# Autodesk Inventor assembly: inner
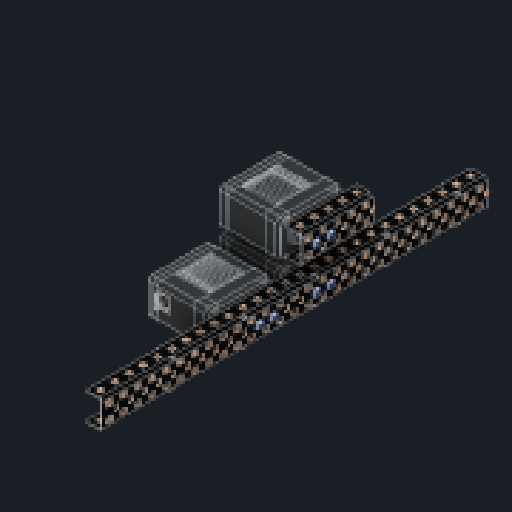
[picture p0: Inventor's stored thumbnail of the model, 512x512]
Saved by Autodesk Inventor 2024 (Build 280153000, 153)
## iProperties
Created: 2024-03-11
Part Number: inner
Document SubType Name: Assembly
Designer: Averey Ku
Author: Averey Ku
## Documents named in this file (17)
- D:\vex_robotics\hardware\cad\eca\chassis\drivebay\inner.iam
- D:\vex_robotics\hardware\cad\VEX-CAD-Inventor-1.41\Structure\C Channel\Aluminum 1x2x1\Alu C 1x2x1x27.ipt
- D:\vex_robotics\hardware\cad\VEX-CAD-Inventor-1.41\Structure\C Channel\Aluminum 1x2x1\Alu C 1x2x1x5.ipt
- D:\vex_robotics\hardware\cad\VEX-CAD-Inventor-1.41\Electronics\Motors with Screws\SteelM-StarS.iam
- D:\vex_robotics\hardware\cad\VEX-CAD-Inventor-1.41\Electronics\Motors with Screws.iam
- D:\vex_robotics\hardware\cad\VEX-CAD-Inventor-1.41\Structure\Hardware\Nut Thin Nylock.ipt
- D:\vex_robotics\hardware\cad\VEX-CAD-Inventor-1.41\Structure\Hardware\Screw Steel - Star\SScrew Star Smooth 1.500.ipt
- D:\vex_robotics\hardware\cad\VEX-CAD-Inventor-1.41\Structure\Hardware\Screw Steel - Star.ipt
- D:\vex_robotics\hardware\cad\VEX-CAD-Inventor-1.41\Structure\Standoff\Standoff .50.ipt
- D:\vex_robotics\hardware\cad\VEX-CAD-Inventor-1.41\Structure\Standoff.ipt
- D:\vex_robotics\hardware\cad\VEX-CAD-Inventor-1.41\Structure\Hardware\Screw Steel - Star\SScrew Star Smooth 1.250.ipt
- D:\vex_robotics\hardware\cad\VEX-CAD-Inventor-1.41\Motion\Spacers\Spacer Nylon .500 OD\NSpacer Black .500 OD x .500.ipt
- D:\vex_robotics\hardware\cad\VEX-CAD-Inventor-1.41\Motion\Spacers\Spacer Nylon .500 OD.ipt
- D:\vex_robotics\hardware\cad\VEX-CAD-Inventor-1.41\Structure\Hardware\Screw Steel - Star\SScrew Star Smooth 1.750.ipt
- D:\vex_robotics\hardware\cad\hardware\.375 OD Aluminum Spacer 0.875.ipt
- D:\vex_robotics\hardware\cad\VEX-CAD-Inventor-1.41\Structure\Hardware\Screw Shoulder Robosource\SScrew Shoulder Smooth .375 x .12.ipt
- D:\vex_robotics\hardware\cad\VEX-CAD-Inventor-1.41\Structure\Hardware\Screw Shoulder Robosource.ipt
## Components (17 placed, 11 different names)
1. Alu C 1x2x1x27:1 — Insert:1, Mate:1, Insert:3, Mate:3, Insert:4, Mate:4, Insert:8, Insert:9, Insert:10, Insert:11, Insert:12, Insert:13, Insert:14
2. Alu C 1x2x1x5:1 — Insert:1, Mate:1, Insert:2, Mate:2, Insert:5, Insert:6, Insert:7, Insert:15, Insert:16
3. SteelM-StarS:1 [sub-assembly] — Insert:4, Mate:4
4. SteelM-StarS:2 [sub-assembly] — Insert:3, Mate:3
5. SteelM-StarS:3 [sub-assembly] — Insert:2, Mate:2
6. Nut Thin Nylock:1 — Insert:5
7. Nut Thin Nylock:2 — Insert:6
8. SScrew Star Smooth 1.500:1 — Insert:7
9. Standoff .50:1 — Insert:8
10. SScrew Star Smooth 1.250:2 — Insert:11
11. Nut Thin Nylock:3 — Insert:9
12. Nut Thin Nylock:4 — Insert:10
13. NSpacer Black .500 OD x .500:1 — Insert:14
14. SScrew Star Smooth 1.750:3 — Insert:13
15. Nut Thin Nylock:5 — Insert:15
16. .375 OD Aluminum Spacer 0.875:1 — Insert:12
17. SScrew Shoulder Smooth .375 x .12:1 — Insert:16
## Relationships (20: Insert 16, Mate 4)
- Insert:1 (12.7 mm): Alu C 1x2x1x27:1 ↔ Alu C 1x2x1x5:1
- Mate:1: Alu C 1x2x1x27:1 ↔ Alu C 1x2x1x5:1
- Insert:2: Alu C 1x2x1x5:1 ↔ SteelM-StarS:3
- Mate:2: Alu C 1x2x1x5:1 ↔ SteelM-StarS:3
- Insert:3: Alu C 1x2x1x27:1 ↔ SteelM-StarS:2
- Mate:3: Alu C 1x2x1x27:1 ↔ SteelM-StarS:2
- Insert:4: Alu C 1x2x1x27:1 ↔ SteelM-StarS:1
- Mate:4: Alu C 1x2x1x27:1 ↔ SteelM-StarS:1
- Insert:5: Alu C 1x2x1x5:1 ↔ Nut Thin Nylock:1
- Insert:6: Alu C 1x2x1x5:1 ↔ Nut Thin Nylock:2
- Insert:7 (6.35 mm): Alu C 1x2x1x5:1 ↔ SScrew Star Smooth 1.500:1
- Insert:8: Alu C 1x2x1x27:1 ↔ Standoff .50:1
- Insert:9: Alu C 1x2x1x27:1 ↔ Nut Thin Nylock:3
- Insert:10: Alu C 1x2x1x27:1 ↔ Nut Thin Nylock:4
- Insert:11: Alu C 1x2x1x27:1 ↔ SScrew Star Smooth 1.250:2
- Insert:12: Alu C 1x2x1x27:1 ↔ .375 OD Aluminum Spacer 0.875:1
- Insert:13: Alu C 1x2x1x27:1 ↔ SScrew Star Smooth 1.750:3
- Insert:14: Alu C 1x2x1x27:1 ↔ NSpacer Black .500 OD x .500:1
- Insert:15: Alu C 1x2x1x5:1 ↔ Nut Thin Nylock:5
- Insert:16: Alu C 1x2x1x5:1 ↔ SScrew Shoulder Smooth .375 x .12:1
